# Autodesk Inventor assembly: 中间洞四方轴套
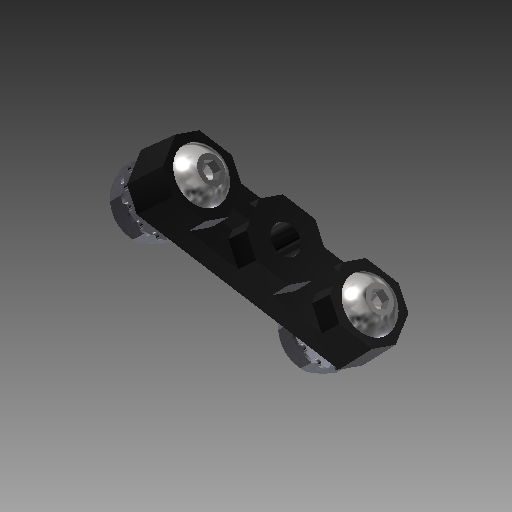
[picture p0: Inventor's stored thumbnail of the model, 512x512]
Saved by Autodesk Inventor 2019.3 (Build 233278000, 278)
## iProperties
Created: 2018-09-04
Part Number: 中间洞四方轴套
Material: 常规
Document SubType Name: Assembly
Designer: aresp
Mass: 8.20296 g
Surface Area: 29.2574 cm^2
Volume: 2.34608 cm^3
Density: 3.49645 g/cm^3
d1_d2: 0.000 mm
Author: aresp
## Documents named in this file (3)
- D:\cad\零件库\中间洞四方轴套.iam
- D:\cad\零件库\三号螺丝+螺帽套.iam
- D:\cad\零件库\垫片轴套大白等\Bearing Flat.ipt
## Components (3 placed, 2 different names)
1. 三号螺丝+螺帽套:1 [sub-assembly]
2. 三号螺丝+螺帽套:2 [sub-assembly]
3. Bearing Flat:1
## Named parameters: d1_d2 = 0 mm
